# Autodesk Inventor assembly: Wózek_inwalidzki
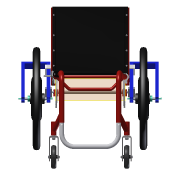
[picture p0: Inventor's stored thumbnail of the model, 180x180]
Saved by Autodesk Inventor 2015 (Build 190159000, 159)
## iProperties
Created: 2016-01-12
Part Number: Wózek_inwalidzki
Document SubType Name: Assembly
Designer: graaapsik
Author: graaapsik
## Documents named in this file (31)
- C:\Users\EriveltonDell\Documents\Centro Universitário da FEI\Wheelchair\CADEIRA DE RODAS - DESENHO\GITHUB\Montagem com Garfo Retangular.iam
- C:\Users\EriveltonDell\Documents\Centro Universitário da FEI\Wheelchair\CADEIRA DE RODAS - DESENHO\GITHUB\Hamulec.iam
- C:\Users\EriveltonDell\Documents\Centro Universitário da FEI\Wheelchair\CADEIRA DE RODAS - DESENHO\GITHUB\Koło_przednie.iam
- C:\Users\EriveltonDell\Documents\Centro Universitário da FEI\Wheelchair\CADEIRA DE RODAS - DESENHO\GITHUB\Rama_wozka.iam
- C:\Users\EriveltonDell\Documents\Centro Universitário da FEI\Wheelchair\CADEIRA DE RODAS - DESENHO\GITHUB\Tapicerka_oparcia.iam
- C:\Users\EriveltonDell\Documents\Centro Universitário da FEI\Wheelchair\CADEIRA DE RODAS - DESENHO\GITHUB\Tapicerka_siedziska.iam
- C:\Users\EriveltonDell\Documents\Centro Universitário da FEI\Wheelchair\CADEIRA DE RODAS - DESENHO\GITHUB\Ciąg.iam
- C:\Users\EriveltonDell\Documents\Centro Universitário da FEI\Wheelchair\CADEIRA DE RODAS - DESENHO\GITHUB\Widelec.iam
- C:\Users\EriveltonDell\Documents\Centro Universitário da FEI\Wheelchair\CADEIRA DE RODAS - DESENHO\GITHUB\Zaślepka_do_widelca.ipt
- C:\Users\EriveltonDell\Documents\Centro Universitário da FEI\Wheelchair\CADEIRA DE RODAS - DESENHO\GITHUB\Podnóżek.iam
- C:\Users\EriveltonDell\Documents\Centro Universitário da FEI\Wheelchair\CADEIRA DE RODAS - DESENHO\GITHUB\Zaślepka_do_rur_fi32.ipt
- C:\Users\EriveltonDell\Documents\Centro Universitário da FEI\Wheelchair\CADEIRA DE RODAS - DESENHO\GITHUB\suporte-rodas-esq.ipt
- C:\Users\EriveltonDell\Documents\Centro Universitário da FEI\Wheelchair\CADEIRA DE RODAS - DESENHO\GITHUB\suporte-rodas.ipt
- C:\Users\EriveltonDell\Documents\Centro Universitário da FEI\Wheelchair\CADEIRA DE RODAS - DESENHO\GITHUB\suporte-eixo.ipt
- C:\Users\EriveltonDell\Documents\Centro Universitário da FEI\Wheelchair\CADEIRA DE RODAS - DESENHO\GITHUB\Barra-garfo.ipt
- C:\Users\EriveltonDell\Documents\Centro Universitário da FEI\Wheelchair\CADEIRA DE RODAS - DESENHO\GITHUB\suporte-eixo - 2.ipt
- C:\Users\EriveltonDell\Documents\Centro Universitário da FEI\Wheelchair\CADEIRA DE RODAS - DESENHO\GITHUB\ISO 4032 - M12ISO.ipt
- C:\Users\EriveltonDell\Documents\Centro Universitário da FEI\Wheelchair\CADEIRA DE RODAS - DESENHO\GITHUB\ISO 4032 - M8ISO.ipt
- C:\Users\EriveltonDell\Documents\Centro Universitário da FEI\Wheelchair\CADEIRA DE RODAS - DESENHO\GITHUB\GARFO - Copy.ipt
- C:\Users\EriveltonDell\Documents\Centro Universitário da FEI\Wheelchair\CADEIRA DE RODAS - DESENHO\GITHUB\suporte-barra - Copy.ipt
- C:\Users\EriveltonDell\Documents\Centro Universitário da FEI\Wheelchair\CADEIRA DE RODAS - DESENHO\GITHUB\edge.ipt
- C:\Users\EriveltonDell\Documents\Centro Universitário da FEI\Wheelchair\CADEIRA DE RODAS - DESENHO\GITHUB\motorEaro.iam
- C:\Users\EriveltonDell\Documents\Centro Universitário da FEI\Wheelchair\CADEIRA DE RODAS - DESENHO\GITHUB\Imported Components\Hub_Motor_MagicPie2_ASM\Hub_Motor_MagicPie2_ASM.iam
- C:\Users\EriveltonDell\Documents\Centro Universitário da FEI\Wheelchair\CADEIRA DE RODAS - DESENHO\GITHUB\Barra-superior.ipt
- C:\Users\EriveltonDell\Documents\Centro Universitário da FEI\Wheelchair\CADEIRA DE RODAS - DESENHO\GITHUB\pino.ipt
- C:\Users\EriveltonDell\Documents\Centro Universitário da FEI\Wheelchair\CADEIRA DE RODAS - DESENHO\GITHUB\Chapa Pino.ipt
- C:\Users\EriveltonDell\Documents\Centro Universitário da FEI\Wheelchair\CADEIRA DE RODAS - DESENHO\GITHUB\Chapa Pino comp.ipt
- C:\Users\EriveltonDell\Documents\Centro Universitário da FEI\Wheelchair\CADEIRA DE RODAS - DESENHO\GITHUB\suporte-barra - tampa.ipt
- C:\Users\EriveltonDell\Documents\Centro Universitário da FEI\Wheelchair\CADEIRA DE RODAS - DESENHO\GITHUB\Abraca estrutura.ipt
- C:\Users\EriveltonDell\Documents\Centro Universitário da FEI\Wheelchair\CADEIRA DE RODAS - DESENHO\GITHUB\Abraca estrutura - comp.ipt
- C:\Users\EriveltonDell\Documents\Centro Universitário da FEI\Wheelchair\CADEIRA DE RODAS - DESENHO\GITHUB\Abraca estrutura - 20.ipt
## Components (58 placed, 30 different names)
1. Rama_wozka:1 [sub-assembly] — Zestawiający:7, Zestawiający:8, Zestawiający:9, Zestawiający:10, Zestawiający:11, Zestawiający:12, Równoległy:1, Zestawiający:15, Symetria:1, Równoległy:2, Zestawiający:20, Zestawiający:22, Zestawiający:27, Zestawiający:29, Zestawiający:36, Zestawiający:37, Równoległy:3, Zestawiający:38, Zestawiający:39, Zestawiający:40, Zestawiający:41, Zestawiający:42, Zestawiający:43, Zestawiający:44, Zestawiający:45, Angle:9, Insert:13, Insert:14, Angle:12, Insert:30, Insert:31, Mate:143, Mate:144, Mate:145, Mate:147
2. Ciąg:1 [sub-assembly]
3. Ciąg:2 [sub-assembly]
4. Widelec:1 [sub-assembly] — Zestawiający:9, Zestawiający:11, Wstaw:3
5. Widelec:2 [sub-assembly] — Zestawiający:10, Zestawiający:12, Zestawiający:13, Zestawiający:14, Symetria:1
6. Koło_przednie:1 [sub-assembly] — Wstaw:3
7. Koło_przednie:2 [sub-assembly] — Zestawiający:13, Zestawiający:14
8. Hamulec:1 [sub-assembly] — Zestawiający:38, Zestawiający:39, Angle:9
9. Tapicerka_oparcia:1 [sub-assembly] — Równoległy:1, Zestawiający:16
10. Tapicerka_siedziska:1 [sub-assembly] — Zestawiający:15, Zestawiający:16, Angle:10, Angle:11
11. Zaślepka_do_widelca:1 — Zestawiający:8, Zestawiający:45
12. Zaślepka_do_widelca:2 — Zestawiający:7, Zestawiający:44
13. Podnóżek:1 [sub-assembly] — Zestawiający:36, Zestawiający:37, Równoległy:3
14. Zaślepka_do_rur_fi32:1 — Zestawiający:22, Zestawiający:42
15. Zaślepka_do_rur_fi32:2 — Zestawiający:27, Zestawiający:40
16. Zaślepka_do_rur_fi32:3 — Zestawiający:20, Zestawiający:43
17. Zaślepka_do_rur_fi32:5 — Zestawiający:29, Zestawiający:41
18. suporte-rodas-esq:1 — Insert:14, Angle:10, Mate:55, Tangent:19, Tangent:20
19. suporte-rodas:1 — Insert:13, Angle:11, Mate:62, Tangent:21, Tangent:22
20. suporte-eixo:2 — Mate:55, Tangent:19, Tangent:20
21. Barra-garfo:1 — Angle:12, Mate:79, Mate:90, Mate:91, Insert:32, Mate:135, Mate:136, Mate:138, Mate:140
22. suporte-eixo - 2:1 — Mate:62, Tangent:21, Tangent:22, Mate:118
23. Zaślepka_do_rur_fi32:6 — Insert:30
24. Zaślepka_do_rur_fi32:7 — Insert:31
25. ISO 4032 M12:1
26. ISO 4032 M8:1
27. ISO 4032 M8:3
28. GARFO - Copy:1 — Mate:80, Mate:81, Flush:5, Flush:6, Mate:94, Mate:95, Mate:96, Mate:97, Mate:98, Mate:113, Mate:114, Flush:10, Mate:122, Mate:129, Mate:131, Mate:134
29. GARFO - Copy:2 — Flush:5, Mate:88, Mate:99, Mate:100, Mate:101, Mate:102, Flush:7, Flush:8, Mate:112, Mate:115, Mate:116, Mate:119, Flush:9, Mate:120, Mate:124, Angle:13, Mate:126, Mate:133
30. suporte-barra - Copy:2 — Mate:79, Mate:80, Mate:81, Insert:32, Flush:15, Flush:16, Mate:139
31. suporte-barra - Copy:3 — Mate:88, Mate:90, Mate:91, Flush:13, Flush:14, Angle:14, Mate:137
32. edge:1 — Flush:6, Mate:94, Mate:95
33. edge:2 — Mate:96, Mate:97, Mate:98
34. edge:3 — Mate:101, Mate:102, Flush:7
35. edge:4 — Mate:99, Mate:100, Flush:8
36. Ciąg:3 [sub-assembly]
37. motorEaro:1 [sub-assembly] — Mate:112
38. Hub_Motor_MagicPie2_ASM:2 [sub-assembly] — Mate:113, Mate:114, Mate:117
39. Hub_Motor_MagicPie2_ASM:3 [sub-assembly] — Mate:115, Mate:116, Mate:117
40. Barra-superior:1 — Mate:118, Mate:119, Mate:121, Mate:123
41. pino:1 — Flush:9, Mate:120, Mate:121, Mate:125, Mate:127
42. pino:2 — Flush:10, Mate:122, Mate:123, Mate:130, Mate:132
43. Chapa Pino:1 — Mate:124, Mate:125, Angle:13, Mate:128
44. Chapa Pino comp:1 — Mate:126, Mate:127, Mate:128, Flush:11
45. Chapa Pino:2 — Mate:129, Mate:130, Flush:11, Flush:12
46. Chapa Pino comp:2 — Mate:131, Mate:132, Flush:12
47. suporte-barra - tampa:1 — Mate:133, Flush:13, Flush:14
48. suporte-barra - tampa:2 — Mate:134, Flush:15, Flush:16
49. Abraca estrutura:1 — Mate:135, Angle:14, Flush:17, Flush:18, Mate:137, Flush:19
50. Abraca estrutura:2 — Mate:136, Flush:17, Flush:18, Mate:141, Flush:22, Flush:23
51. Abraca estrutura:3 — Mate:138, Flush:19, Mate:139, Flush:20, Flush:21
52. Abraca estrutura:4 — Mate:140, Flush:20, Flush:21, Mate:142, Flush:24
53. Abraca estrutura - comp:1 — Mate:141, Flush:22, Flush:23, Angle:15, Flush:31, Flush:32
54. Abraca estrutura - comp:2 — Mate:142, Flush:24, Mate:146, Flush:28, Flush:31
55. Abraca estrutura - 20:1 — Mate:143, Angle:15, Flush:26, Flush:27, Flush:32
56. Abraca estrutura - 20:2 — Mate:144, Flush:26, Flush:27
57. Abraca estrutura - 20:3 — Mate:145, Mate:146, Flush:28, Flush:29, Flush:30
58. Abraca estrutura - 20:4 — Mate:147, Flush:29, Flush:30
## Relationships (125: Mate 77, Flush 30, Angle 7, Insert 6, Tangent 4, Symmetry 1)
- Zestawiający:7 [Mate]: Rama_wozka:1 ↔ Zaślepka_do_widelca:2
- Zestawiający:8 [Mate]: Rama_wozka:1 ↔ Zaślepka_do_widelca:1
- Zestawiający:9 [Mate]: Rama_wozka:1 ↔ Widelec:1
- Zestawiający:10 [Mate]: Rama_wozka:1 ↔ Widelec:2
- Zestawiający:11 [Mate]: Rama_wozka:1 ↔ Widelec:1
- Zestawiający:12 [Mate]: Rama_wozka:1 ↔ Widelec:2
- Zestawiający:13 [Mate]: Widelec:2 ↔ Koło_przednie:2
- Zestawiający:14 [Mate]: Widelec:2 ↔ Koło_przednie:2
- Równoległy:1 [Flush] (-16 mm): Rama_wozka:1 ↔ Tapicerka_oparcia:1
- Zestawiający:15 [Mate] (16 mm): Rama_wozka:1 ↔ Tapicerka_siedziska:1
- Zestawiający:16 [Mate] (0.25 mm): Tapicerka_oparcia:1 ↔ Tapicerka_siedziska:1
- Symetria:1 [Symmetry]: Rama_wozka:1 ↔ Widelec:2
- Równoległy:2 [Flush]: Rama_wozka:1
- Zestawiający:20 [Mate]: Rama_wozka:1 ↔ Zaślepka_do_rur_fi32:3
- Zestawiający:22 [Mate]: Rama_wozka:1 ↔ Zaślepka_do_rur_fi32:1
- Zestawiający:27 [Mate]: Rama_wozka:1 ↔ Zaślepka_do_rur_fi32:2
- Zestawiający:29 [Mate]: Rama_wozka:1 ↔ Zaślepka_do_rur_fi32:5
- Wstaw:3 [Insert]: Widelec:1 ↔ Koło_przednie:1
- Zestawiający:36 [Mate]: Rama_wozka:1 ↔ Podnóżek:1
- Zestawiający:37 [Mate]: Rama_wozka:1 ↔ Podnóżek:1
- Równoległy:3 [Flush] (150 mm): Rama_wozka:1 ↔ Podnóżek:1
- Zestawiający:38 [Mate]: Rama_wozka:1 ↔ Hamulec:1
- Zestawiający:39 [Mate] (40 mm): Rama_wozka:1 ↔ Hamulec:1
- Zestawiający:40 [Mate]: Rama_wozka:1 ↔ Zaślepka_do_rur_fi32:2
- Zestawiający:41 [Mate]: Rama_wozka:1 ↔ Zaślepka_do_rur_fi32:5
- Zestawiający:42 [Mate]: Rama_wozka:1 ↔ Zaślepka_do_rur_fi32:1
- Zestawiający:43 [Mate]: Rama_wozka:1 ↔ Zaślepka_do_rur_fi32:3
- Zestawiający:44 [Mate]: Rama_wozka:1 ↔ Zaślepka_do_widelca:2
- Zestawiający:45 [Mate]: Rama_wozka:1 ↔ Zaślepka_do_widelca:1
- Angle:9 (0 deg): Rama_wozka:1 ↔ Hamulec:1
- Insert:13 (150 mm): Rama_wozka:1 ↔ suporte-rodas:1
- Insert:14 (150 mm): Rama_wozka:1 ↔ suporte-rodas-esq:1
- Angle:10 (90 deg): Tapicerka_siedziska:1 ↔ suporte-rodas-esq:1
- Angle:11 (90 deg): Tapicerka_siedziska:1 ↔ suporte-rodas:1
- Mate:55: suporte-rodas-esq:1 ↔ suporte-eixo:2
- Tangent:19: suporte-rodas-esq:1 ↔ suporte-eixo:2
- Tangent:20: suporte-rodas-esq:1 ↔ suporte-eixo:2
- Angle:12 (0 deg): Rama_wozka:1 ↔ Barra-garfo:1
- Mate:62: suporte-rodas:1 ↔ suporte-eixo - 2:1
- Tangent:21: suporte-rodas:1 ↔ suporte-eixo - 2:1
- Tangent:22: suporte-rodas:1 ↔ suporte-eixo - 2:1
- Insert:30 (-8 mm): Rama_wozka:1 ↔ Zaślepka_do_rur_fi32:6
- Insert:31 (-8 mm): Rama_wozka:1 ↔ Zaślepka_do_rur_fi32:7
- Mate:79: Barra-garfo:1 ↔ suporte-barra - Copy:2
- Mate:80: GARFO - Copy:1 ↔ suporte-barra - Copy:2
- Mate:81: GARFO - Copy:1 ↔ suporte-barra - Copy:2
- Flush:5: GARFO - Copy:1 ↔ GARFO - Copy:2
- Mate:88: GARFO - Copy:2 ↔ suporte-barra - Copy:3
- Mate:90: Barra-garfo:1 ↔ suporte-barra - Copy:3
- Mate:91: Barra-garfo:1 ↔ suporte-barra - Copy:3
- Flush:6: GARFO - Copy:1 ↔ edge:1
- Mate:94: GARFO - Copy:1 ↔ edge:1
- Mate:95: GARFO - Copy:1 ↔ edge:1
- Mate:96: GARFO - Copy:1 ↔ edge:2
- Mate:97: GARFO - Copy:1 ↔ edge:2
- Mate:98: GARFO - Copy:1 ↔ edge:2
- Mate:99: GARFO - Copy:2 ↔ edge:4
- Mate:100: GARFO - Copy:2 ↔ edge:4
- Mate:101: GARFO - Copy:2 ↔ edge:3
- Mate:102: GARFO - Copy:2 ↔ edge:3
- Flush:7: GARFO - Copy:2 ↔ edge:3
- Flush:8: GARFO - Copy:2 ↔ edge:4
- Insert:32: Barra-garfo:1 ↔ suporte-barra - Copy:2
- Mate:112: GARFO - Copy:2 ↔ motorEaro:1
- Mate:113: GARFO - Copy:1 ↔ Hub_Motor_MagicPie2_ASM:2
- Mate:114: GARFO - Copy:1 ↔ Hub_Motor_MagicPie2_ASM:2
- Mate:115: GARFO - Copy:2 ↔ Hub_Motor_MagicPie2_ASM:3
- Mate:116: GARFO - Copy:2 ↔ Hub_Motor_MagicPie2_ASM:3
- Mate:117: Hub_Motor_MagicPie2_ASM:2 ↔ Hub_Motor_MagicPie2_ASM:3
- Mate:118: suporte-eixo - 2:1 ↔ Barra-superior:1
- Mate:119 (14 mm): GARFO - Copy:2 ↔ Barra-superior:1
- Flush:9: GARFO - Copy:2 ↔ pino:1
- Mate:120: GARFO - Copy:2 ↔ pino:1
- Mate:121: Barra-superior:1 ↔ pino:1
- Flush:10: GARFO - Copy:1 ↔ pino:2
- Mate:122: GARFO - Copy:1 ↔ pino:2
- Mate:123: Barra-superior:1 ↔ pino:2
- Mate:124: GARFO - Copy:2 ↔ Chapa Pino:1
- Mate:125: pino:1 ↔ Chapa Pino:1
- Angle:13 (90 deg): GARFO - Copy:2 ↔ Chapa Pino:1
- Mate:126: GARFO - Copy:2 ↔ Chapa Pino comp:1
- Mate:127: pino:1 ↔ Chapa Pino comp:1
- Mate:128: Chapa Pino:1 ↔ Chapa Pino comp:1
- Mate:129: GARFO - Copy:1 ↔ Chapa Pino:2
- Mate:130: pino:2 ↔ Chapa Pino:2
- Flush:11: Chapa Pino comp:1 ↔ Chapa Pino:2
- Mate:131: GARFO - Copy:1 ↔ Chapa Pino comp:2
- Mate:132: pino:2 ↔ Chapa Pino comp:2
- Flush:12: Chapa Pino:2 ↔ Chapa Pino comp:2
- Mate:133: GARFO - Copy:2 ↔ suporte-barra - tampa:1
- Flush:13: suporte-barra - Copy:3 ↔ suporte-barra - tampa:1
- Flush:14: suporte-barra - Copy:3 ↔ suporte-barra - tampa:1
- Mate:134: GARFO - Copy:1 ↔ suporte-barra - tampa:2
- Flush:15: suporte-barra - Copy:2 ↔ suporte-barra - tampa:2
- Flush:16: suporte-barra - Copy:2 ↔ suporte-barra - tampa:2
- Mate:135: Barra-garfo:1 ↔ Abraca estrutura:1
- Angle:14 (85 deg): suporte-barra - Copy:3 ↔ Abraca estrutura:1
- Mate:136: Barra-garfo:1 ↔ Abraca estrutura:2
- Flush:17: Abraca estrutura:1 ↔ Abraca estrutura:2
- Flush:18: Abraca estrutura:1 ↔ Abraca estrutura:2
- Mate:137 (75 mm): suporte-barra - Copy:3 ↔ Abraca estrutura:1
- Mate:138: Barra-garfo:1 ↔ Abraca estrutura:3
- Flush:19: Abraca estrutura:1 ↔ Abraca estrutura:3
- Mate:139 (75 mm): suporte-barra - Copy:2 ↔ Abraca estrutura:3
- Mate:140: Barra-garfo:1 ↔ Abraca estrutura:4
- Flush:20: Abraca estrutura:3 ↔ Abraca estrutura:4
- Flush:21: Abraca estrutura:3 ↔ Abraca estrutura:4
- Mate:141: Abraca estrutura:2 ↔ Abraca estrutura - comp:1
- Flush:22: Abraca estrutura:2 ↔ Abraca estrutura - comp:1
- Flush:23 (-10 mm): Abraca estrutura:2 ↔ Abraca estrutura - comp:1
- Mate:142: Abraca estrutura:4 ↔ Abraca estrutura - comp:2
- Flush:24: Abraca estrutura:4 ↔ Abraca estrutura - comp:2
- Mate:143: Rama_wozka:1 ↔ Abraca estrutura - 20:1
- Angle:15 (0 deg): Abraca estrutura - comp:1 ↔ Abraca estrutura - 20:1
- Mate:144: Rama_wozka:1 ↔ Abraca estrutura - 20:2
- Flush:26: Abraca estrutura - 20:1 ↔ Abraca estrutura - 20:2
- Flush:27: Abraca estrutura - 20:1 ↔ Abraca estrutura - 20:2
- Mate:145: Rama_wozka:1 ↔ Abraca estrutura - 20:3
- Mate:146: Abraca estrutura - comp:2 ↔ Abraca estrutura - 20:3
- Flush:28: Abraca estrutura - comp:2 ↔ Abraca estrutura - 20:3
- Mate:147: Rama_wozka:1 ↔ Abraca estrutura - 20:4
- Flush:29: Abraca estrutura - 20:3 ↔ Abraca estrutura - 20:4
- Flush:30: Abraca estrutura - 20:3 ↔ Abraca estrutura - 20:4
- Flush:31: Abraca estrutura - comp:1 ↔ Abraca estrutura - comp:2
- Flush:32: Abraca estrutura - comp:1 ↔ Abraca estrutura - 20:1
## Named parameters: sa_0 = 1.6e-12, sa_1 = -6.84e-11, sa_2 = -70000
note: some values were not read from the file. Shown as the stored number, unit unknown: "sa_0", "sa_1", "sa_2".
